# Autodesk Inventor assembly: assembly crankshaft
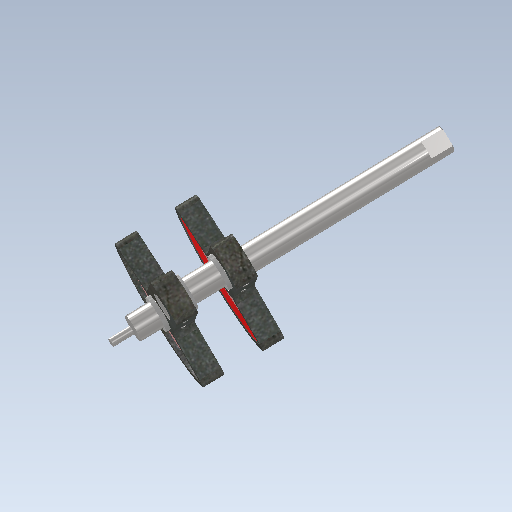
[picture p0: Inventor's stored thumbnail of the model, 512x512]
Saved by Autodesk Inventor 2020 (Build 240168000, 168)
## iProperties
Created: 2021-07-04
Part Number: assembly crankshaft
Document SubType Name: Assembly
Designer: lokes
Author: lokes
## Documents named in this file (6)
- C:\Users\lokes\OneDrive\Desktop\major\assembly crankshaft.iam
- C:\Users\lokes\OneDrive\Desktop\major\CRANKSHAFT.ipt
- C:\Users\lokes\OneDrive\Desktop\major\crankshaft counterweight.ipt
- C:\Users\lokes\OneDrive\Desktop\major\crankshaft pin.ipt
- C:\Users\lokes\OneDrive\Desktop\major\CRANKSHAFT VALVE CRANK.ipt
- C:\Users\lokes\OneDrive\Documents\Inventor\Content Center Files\R2020\en-US\ISO 2338(2)\ISO 2338 - 3 h8 x 20.ipt
## Components (9 placed, 5 different names)
1. CRANKSHAFT:1 — Mate:1, Mate:2, Mate:9, Mate:16
2. crankshaft counterweight:1 — Mate:1, Mate:2, Mate:3, Mate:4, Mate:9, Mate:14, Mate:15, Mate:17
3. crankshaft pin:1 — Mate:3, Mate:4, Mate:5, Mate:6
4. crankshaft counterweight:2 — Mate:5, Mate:6, Mate:7, Mate:8, Mate:10, Mate:11, Mate:12, Mate:13
5. CRANKSHAFT VALVE CRANK:1 — Mate:7, Mate:8
6. ISO 2338 3 h8 x 20:1 — Mate:14, Mate:15
7. ISO 2338 3 h8 x 20:2 — Mate:16, Mate:17
8. ISO 2338 3 h8 x 20:3 — Mate:12, Mate:13
9. ISO 2338 3 h8 x 20:4 — Mate:10, Mate:11
## Relationships (17: Mate 17)
- Mate:1: CRANKSHAFT:1 ↔ crankshaft counterweight:1
- Mate:2: CRANKSHAFT:1 ↔ crankshaft counterweight:1
- Mate:3: crankshaft counterweight:1 ↔ crankshaft pin:1
- Mate:4: crankshaft counterweight:1 ↔ crankshaft pin:1
- Mate:5: crankshaft pin:1 ↔ crankshaft counterweight:2
- Mate:6: crankshaft pin:1 ↔ crankshaft counterweight:2
- Mate:7: crankshaft counterweight:2 ↔ CRANKSHAFT VALVE CRANK:1
- Mate:8: crankshaft counterweight:2 ↔ CRANKSHAFT VALVE CRANK:1
- Mate:9: CRANKSHAFT:1 ↔ crankshaft counterweight:1
- Mate:10: crankshaft counterweight:2 ↔ ISO 2338 3 h8 x 20:4
- Mate:11: crankshaft counterweight:2 ↔ ISO 2338 3 h8 x 20:4
- Mate:12: crankshaft counterweight:2 ↔ ISO 2338 3 h8 x 20:3
- Mate:13: crankshaft counterweight:2 ↔ ISO 2338 3 h8 x 20:3
- Mate:14: crankshaft counterweight:1 ↔ ISO 2338 3 h8 x 20:1
- Mate:15: crankshaft counterweight:1 ↔ ISO 2338 3 h8 x 20:1
- Mate:16: CRANKSHAFT:1 ↔ ISO 2338 3 h8 x 20:2
- Mate:17: crankshaft counterweight:1 ↔ ISO 2338 3 h8 x 20:2
